# Autodesk Inventor assembly: 045_DP_D_167__F_D_166_3__2_14b
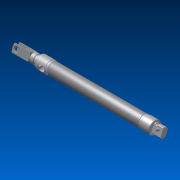
[picture p0: Inventor's stored thumbnail of the model, 180x180]
Saved by Autodesk Inventor 2013 (Build 170138000, 138)
## iProperties
Created: 2013-07-19
Part Number: 045_DP_D_167__F_D_166_3__2_14b
Document SubType Name: Assembly
Designer: nowireless
Author: nowireless
## Documents named in this file (6)
- E:\FRC_Projects\Cad\Inventor_Projects\Shooter_No_Welding\Thrower\cylinder\045_DP_D_167__F_D_166_3__2_14b.iam
- E:\FRC_Projects\Cad\Inventor_Projects\Shooter_No_Welding\Thrower\cylinder\1.ipt
- E:\FRC_Projects\Cad\Inventor_Projects\Shooter_No_Welding\Thrower\cylinder\2.ipt
- E:\FRC_Projects\Cad\Inventor_Projects\Shooter_No_Welding\Thrower\cylinder\3.ipt
- E:\FRC_Projects\Cad\Inventor_Projects\Shooter_No_Welding\Thrower\cylinder\7.ipt
- E:\FRC_Projects\Cad\Inventor_Projects\Shooter_No_Welding\Thrower\cylinder\8.ipt
## Components (5 placed, 5 different names)
1. 1:1 — Mate:10, Mate:12, Mate:13, Mate:14, Insert:1
2. 2:1 — Mate:11, Mate:12, Mate:14, Insert:1, Insert:2
3. 3:1 — Insert:2
4. 7:1 — Mate:7, Flush:1, Mate:10, Mate:11, Mate:13
5. 8:1 — Mate:7, Flush:1
## Relationships (9: Mate 6, Insert 2, Flush 1)
- Mate:7: 7:1 ↔ 8:1
- Flush:1: 7:1 ↔ 8:1
- Mate:10: 1:1 ↔ 7:1
- Mate:11: 2:1 ↔ 7:1
- Mate:12: 1:1 ↔ 2:1
- Mate:13: 1:1 ↔ 7:1
- Mate:14: 1:1 ↔ 2:1
- Insert:1: 1:1 ↔ 2:1
- Insert:2: 2:1 ↔ 3:1
